# Autodesk Inventor assembly: Connessione-D
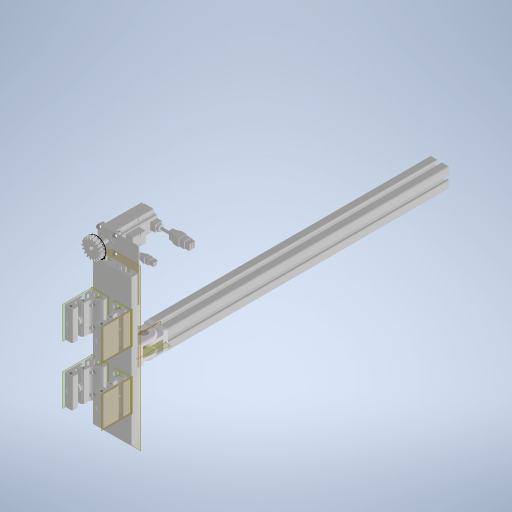
[picture p0: Inventor's stored thumbnail of the model, 512x512]
Saved by Autodesk Inventor 2023 (Build 270158000, 158)
## iProperties
RuleStatus: InUse
Created: 2022-08-22
Part Number: Connessione-D
Document SubType Name: Assembly
Designer: matte
Author: matte
## Documents named in this file (4)
- C:\Users\matte\Documents\GitHub\MDM-CyberOrto-CAD\Dettagli\Connessione-D.iam
- C:\Users\matte\Documents\GitHub\MDM-CyberOrto-CAD\Pezzi singoli\Supporto DX.ipt
- C:\Users\matte\Documents\GitHub\MDM-CyberOrto-CAD\Pezzi singoli\Supporto lineare\Carrello semplice.iam
- C:\Users\matte\Documents\GitHub\MDM-CyberOrto-CAD\Parker components\02-Fasteners\16-Screws\01-Metric Screws\01-Button Head\24-120-8.ipt
## Components (3 placed, 3 different names)
1. Supporto DX:1 — Allineato:6
2. Carrello semplice:1 [sub-assembly] — Allineato:6
3. 24-120-8:1
## Relationships (6: Mate 3, Flush 3)
- [Mate]: Supporto DX:1 ↔ Carrello semplice:1
- [Flush]: Supporto DX:1 ↔ Carrello semplice:1
- [Flush]: Supporto DX:1 ↔ Carrello semplice:1
- [Mate]: Carrello semplice:1 ↔ 24-120-8:1
- [Mate]: Carrello semplice:1 ↔ 24-120-8:1
- Allineato:6 [Flush]: Supporto DX:1 ↔ Carrello semplice:1
